# Autodesk Inventor assembly: pcb_assembled_2
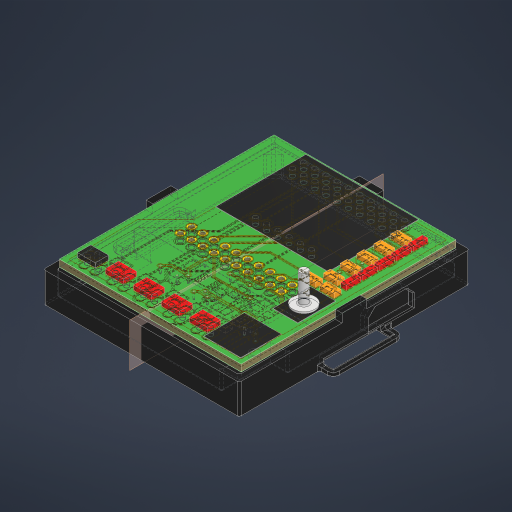
[picture p0: Inventor's stored thumbnail of the model, 512x512]
Saved by Autodesk Inventor 2023 (Build 270158000, 158)
## iProperties
Created: 2022-04-29
Part Number: pcb_assembled_2
Document SubType Name: Assembly
Designer: Haroon Nawaz
Author: Haroon Nawaz
## Documents named in this file (7)
- C:\Users\Haroon Nawaz\Documents\1_Haroon\CE347\git\CE347_Gest\hardware\3D_CAD\pcb_assembled_4.iam
- C:\Users\Haroon Nawaz\Documents\1_Haroon\CE347\git\CE347_Gest\hardware\3D_CAD\pcb_assembled.iam
- C:\Users\Haroon Nawaz\Documents\1_Haroon\CE347\git\CE347_Gest\hardware\3D_CAD\battery.ipt
- C:\Users\Haroon Nawaz\Documents\1_Haroon\CE347\git\CE347_Gest\hardware\3D_CAD\enclosure4.ipt
- C:\Users\Haroon Nawaz\Documents\1_Haroon\CE347\git\CE347_Gest\hardware\3D_CAD\enclosure4_top.ipt
- C:\Users\Haroon Nawaz\Documents\1_Haroon\CE347\git\CE347_Gest\hardware\3D_CAD\enclosure4_button.ipt
- C:\Users\Haroon Nawaz\Documents\1_Haroon\CE347\git\CE347_Gest\hardware\devboard_mainboard\ESP-D1-mini-mainboard v1.ipt
## Components (6 placed, 6 different names)
1. pcb_assembled:1 [sub-assembly] — Mate:1, Flush:1, Flush:2
2. battery:1
3. enclosure4:1 — Mate:1, Flush:1, Flush:2, Flush:3, Flush:4
4. enclosure4_top:1 — Flush:3, Flush:4, Mate:2
5. enclosure4_button:1 — Mate:2
6. ESP-D1-mini-mainboard v1:1
## Relationships (6: Flush 4, Mate 2)
- Mate:1: pcb_assembled:1 ↔ enclosure4:1
- Flush:1 (1.5 mm): pcb_assembled:1 ↔ enclosure4:1
- Flush:2 (1.5 mm): pcb_assembled:1 ↔ enclosure4:1
- Flush:3: enclosure4:1 ↔ enclosure4_top:1
- Flush:4: enclosure4:1 ↔ enclosure4_top:1
- Mate:2: enclosure4_top:1 ↔ enclosure4_button:1
